# Autodesk Inventor assembly: Chess Assembly
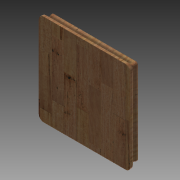
[picture p0: Inventor's stored thumbnail of the model, 180x180]
Saved by Autodesk Inventor 2015 SP1 (Build 190203100, 203)
## iProperties
Created: 2015-06-11
Part Number: Chess Assembly
Document SubType Name: Assembly
Designer: Nathan
Author: Nathan
## Documents named in this file (4)
- X:\1. Nathan Projects\1. General projects\Chess\Chess Assembly.iam
- X:\1. Nathan Projects\1. General projects\Chess\Board Piece 1.ipt
- X:\1. Nathan Projects\1. General projects\Chess\Board Piece 2.ipt
- C:\Users\Nathan\AppData\Local\Autodesk\Autodesk Sync\Cloud\nathan.kirton@gmail.com\1. Nathan Projects\1. General projects\Chess\Outer Rim.ipt
## Components (4 placed, 3 different names)
1. Board Piece 1:1 — Flush:1, Mate:1, Mate:2, Mate:4, Mate:5
2. Board Piece 1:2 — Flush:1, Mate:1, Mate:2, Mate:3
3. Board Piece 2:1 — Mate:3, Mate:4, Mate:5, Mate:6, Mate:7, Mate:8
4. Outer Rim:1 — Mate:6, Mate:7, Mate:8
## Relationships (9: Mate 8, Flush 1)
- Flush:1: Board Piece 1:1 ↔ Board Piece 1:2
- Mate:1: Board Piece 1:1 ↔ Board Piece 1:2
- Mate:2: Board Piece 1:1 ↔ Board Piece 1:2
- Mate:3: Board Piece 1:2 ↔ Board Piece 2:1
- Mate:4: Board Piece 1:1 ↔ Board Piece 2:1
- Mate:5: Board Piece 1:1 ↔ Board Piece 2:1
- Mate:6: Board Piece 2:1 ↔ Outer Rim:1
- Mate:7: Board Piece 2:1 ↔ Outer Rim:1
- Mate:8: Board Piece 2:1 ↔ Outer Rim:1
